# Autodesk Inventor assembly: Adaptationhorizontalachse_obereGabel_Assembly_Rillenkugellager
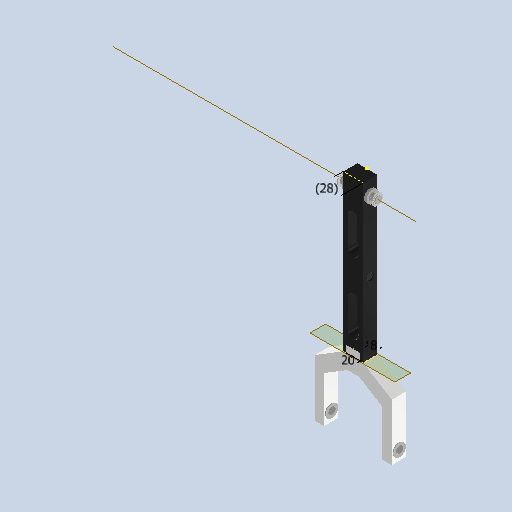
[picture p0: Inventor's stored thumbnail of the model, 512x512]
Saved by Autodesk Inventor 2022 (Build 260153000, 153)
## iProperties
Created: 2022-07-20
Part Number: Adaptationhorizontalachse_obereGabel_Assembly_Rillenkugellager
Document SubType Name: Assembly
Designer: alexw
Mass: 274.315 g
Surface Area: 550.644 cm^2
Volume: 181.539 cm^3
Author: alexw
## Documents named in this file (6)
- C:\Users\AEWALDER\Documents\Inventor\03_CurrentProjects\MasterThesis\PSM_V1_Rillenkugellager\Adaptationhorizontalachse_obereGabel_Assembly_Rillenkugellager.iam
- C:\Users\AEWALDER\Documents\Inventor\03_CurrentProjects\MasterThesis\PSM_V1_Rillenkugellager\SKF_PPMF 101207.ipt
- C:\Users\AEWALDER\Documents\Inventor\03_CurrentProjects\MasterThesis\PSM_V1_Rillenkugellager\ParallelMecha_Gabel_Connection_JointShaft_Rillenkugellager.ipt
- C:\Users\AEWALDER\Documents\Inventor\03_CurrentProjects\MasterThesis\PSM_V1_Rillenkugellager\circlips_din471_10_1.ipt
- C:\Users\AEWALDER\Documents\Inventor\03_CurrentProjects\MasterThesis\PSM_V1_Rillenkugellager\din_988_10_x_16_x_0_10.ipt
- C:\Users\AEWALDER\Documents\Inventor\03_CurrentProjects\MasterThesis\PSM_V1_Rillenkugellager\Adaptationhorizontalachse_Rillenkugellager.ipt
## Components (11 placed, 5 different names)
1. Adaptationhorizontalachse_Rillenkugellager:1 — Passend:1, Passend:2, Fluchtend:1, Passend:21, Passend:22, Passend:23, Passend:24, Passend:25, Passend:26, Passend:27, Passend:28, Einfügen:3, Einfügen:4
2. ParallelMecha_Gabel_Connection_JointShaft_Rillenkugellager:2 — Passend:29, Passend:30, Passend:39, Einfügen:3, Passend:45
3. ParallelMecha_Gabel_Connection_JointShaft_Rillenkugellager:3 — Passend:35, Passend:36, Passend:37, Einfügen:4
4. SKF_PPMF 101207:1 — Passend:27, Passend:28
5. SKF_PPMF 101207:2 — Passend:25, Passend:26
6. SKF_PPMF 101207:3 — Passend:21, Passend:22
7. SKF_PPMF 101207:4 — Passend:23, Passend:24
8. circlips_din471_10_1:1 — Passend:29, Passend:30, Passend:40
9. circlips_din471_10_1:4 — Passend:35, Passend:36, Passend:38
10. din_988_10_x_16_x_0_10:1 — Passend:37, Passend:38
11. din_988_10_x_16_x_0_10:2 — Passend:39, Passend:40
## Relationships (22: Mate 19, Insert 2, Flush 1)
- Passend:1 [Mate]: Adaptationhorizontalachse_Rillenkugellager:1
- Passend:2 [Mate]: Adaptationhorizontalachse_Rillenkugellager:1
- Fluchtend:1 [Flush]: Adaptationhorizontalachse_Rillenkugellager:1
- Passend:21 [Mate]: Adaptationhorizontalachse_Rillenkugellager:1 ↔ SKF_PPMF 101207:3
- Passend:22 [Mate]: Adaptationhorizontalachse_Rillenkugellager:1 ↔ SKF_PPMF 101207:3
- Passend:23 [Mate]: Adaptationhorizontalachse_Rillenkugellager:1 ↔ SKF_PPMF 101207:4
- Passend:24 [Mate]: Adaptationhorizontalachse_Rillenkugellager:1 ↔ SKF_PPMF 101207:4
- Passend:25 [Mate]: Adaptationhorizontalachse_Rillenkugellager:1 ↔ SKF_PPMF 101207:2
- Passend:26 [Mate]: Adaptationhorizontalachse_Rillenkugellager:1 ↔ SKF_PPMF 101207:2
- Passend:27 [Mate]: Adaptationhorizontalachse_Rillenkugellager:1 ↔ SKF_PPMF 101207:1
- Passend:28 [Mate]: Adaptationhorizontalachse_Rillenkugellager:1 ↔ SKF_PPMF 101207:1
- Passend:29 [Mate]: ParallelMecha_Gabel_Connection_JointShaft_Rillenkugellager:2 ↔ circlips_din471_10_1:1
- Passend:30 [Mate]: ParallelMecha_Gabel_Connection_JointShaft_Rillenkugellager:2 ↔ circlips_din471_10_1:1
- Passend:35 [Mate]: ParallelMecha_Gabel_Connection_JointShaft_Rillenkugellager:3 ↔ circlips_din471_10_1:4
- Passend:36 [Mate]: ParallelMecha_Gabel_Connection_JointShaft_Rillenkugellager:3 ↔ circlips_din471_10_1:4
- Passend:37 [Mate]: ParallelMecha_Gabel_Connection_JointShaft_Rillenkugellager:3 ↔ din_988_10_x_16_x_0_10:1
- Passend:38 [Mate]: circlips_din471_10_1:4 ↔ din_988_10_x_16_x_0_10:1
- Passend:39 [Mate]: ParallelMecha_Gabel_Connection_JointShaft_Rillenkugellager:2 ↔ din_988_10_x_16_x_0_10:2
- Passend:40 [Mate]: circlips_din471_10_1:1 ↔ din_988_10_x_16_x_0_10:2
- Einfügen:3 [Insert]: Adaptationhorizontalachse_Rillenkugellager:1 ↔ ParallelMecha_Gabel_Connection_JointShaft_Rillenkugellager:2
- Einfügen:4 [Insert]: Adaptationhorizontalachse_Rillenkugellager:1 ↔ ParallelMecha_Gabel_Connection_JointShaft_Rillenkugellager:3
- Passend:45 [Mate]: ParallelMecha_Gabel_Connection_JointShaft_Rillenkugellager:2
